# Autodesk Inventor assembly: Leg_Feet_Connector_16-10mm_MIR
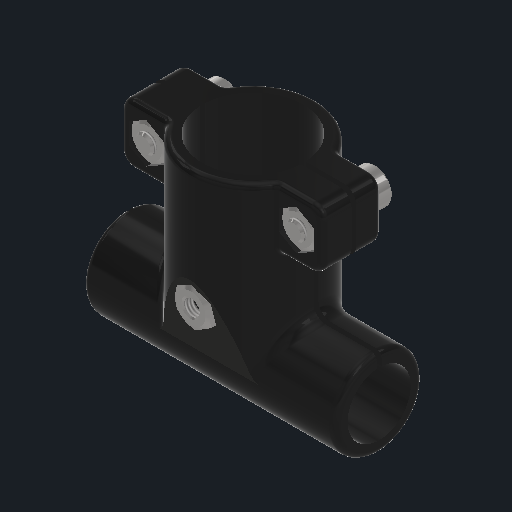
[picture p0: Inventor's stored thumbnail of the model, 512x512]
Saved by Autodesk Inventor 2024.1 (Build 281209000, 209)
## iProperties
Created: 2023-12-04
Part Number: Leg_Feet_Connector_16-10mm_MIR
Document SubType Name: Assembly
Designer: dzw04
Author: dzw04
## Documents named in this file (5)
- C:\Users\dzw04\Saxion\Mechatronica Lectoraat LMECH LED - Database ARG\Component_Database\SARAX\01. CAD\01. 3D_Drawing\02. Sub_Assemblies\Landing_Gear\02. Sub_Assemblies\Leg_Feet_Connector_16-10mm_MIR.iam
- C:\Users\dzw04\Saxion\Mechatronica Lectoraat LMECH LED - Database ARG\Component_Database\SARAX\01. CAD\01. 3D_Drawing\02. Sub_Assemblies\Landing_Gear\01. Parts\Leg_Feet_Connector_16-10mm_MIR.ipt
- C:\Users\dzw04\OneDrive - Saxion\Documenten\Inventor\Content Center Files\R2024\en-US\ISO 4762(2)\ISO 4762 - M3 x 10ISO.ipt
- C:\Users\dzw04\OneDrive - Saxion\Documenten\Inventor\Content Center Files\R2024\en-US\ISO 4035(2)\ISO 4035 - M3 - ISO.ipt
- C:\Users\dzw04\OneDrive - Saxion\Documenten\Inventor\Content Center Files\R2024\en-US\ISO 4762(2)\ISO 4762 - M3 x 16ISO.ipt
## Components (7 placed, 4 different names)
1. Leg_Feet_Connector_16-10mm_MIR:1 — Mate:6, Mate:5, Mate:8, Mate:7, Mate:10, Mate:9, Mate:12, Mate:11, Mate:14, Mate:13, Mate:16, Mate:15
2. ISO 4762 M3 x 10:1 — Mate:6, Mate:5
3. ISO 4035 M3:1 — Mate:8, Mate:7
4. ISO 4762 M3 x 10:2 — Mate:10, Mate:9
5. ISO 4035 M3:2 — Mate:12, Mate:11
6. ISO 4762 M3 x 16:1 — Mate:14, Mate:13
7. ISO 4035 M3:3 — Mate:16, Mate:15
## Relationships (12: Mate 12)
- Mate:6: Leg_Feet_Connector_16-10mm_MIR:1 ↔ ISO 4762 M3 x 10:1
- Mate:5: Leg_Feet_Connector_16-10mm_MIR:1 ↔ ISO 4762 M3 x 10:1
- Mate:8: Leg_Feet_Connector_16-10mm_MIR:1 ↔ ISO 4035 M3:1
- Mate:7: Leg_Feet_Connector_16-10mm_MIR:1 ↔ ISO 4035 M3:1
- Mate:10: Leg_Feet_Connector_16-10mm_MIR:1 ↔ ISO 4762 M3 x 10:2
- Mate:9: Leg_Feet_Connector_16-10mm_MIR:1 ↔ ISO 4762 M3 x 10:2
- Mate:12: Leg_Feet_Connector_16-10mm_MIR:1 ↔ ISO 4035 M3:2
- Mate:11: Leg_Feet_Connector_16-10mm_MIR:1 ↔ ISO 4035 M3:2
- Mate:14: Leg_Feet_Connector_16-10mm_MIR:1 ↔ ISO 4762 M3 x 16:1
- Mate:13: Leg_Feet_Connector_16-10mm_MIR:1 ↔ ISO 4762 M3 x 16:1
- Mate:16: Leg_Feet_Connector_16-10mm_MIR:1 ↔ ISO 4035 M3:3
- Mate:15: Leg_Feet_Connector_16-10mm_MIR:1 ↔ ISO 4035 M3:3
